# Autodesk Inventor assembly: Tube holder 1 assembly
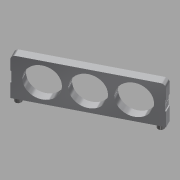
[picture p0: Inventor's stored thumbnail of the model, 180x180]
Saved by Autodesk Inventor 2017 (Build 210142000, 142)
## iProperties
Created: 2017-02-01
Part Number: Tube holder 1 assembly
Document SubType Name: Assembly
Designer: qupec
Author: qupec
## Documents named in this file (4)
- C:\Users\qupec\Desktop\UMD Near Space\RockSat\Renderings and PDFs\Tube holder 1 assembly.iam
- C:\Users\qupec\Documents\Inventor\Content Center Files\R2017\en-US\U UNC 2603(1)\Unbrako - 4 x 1 - 48 - 1 - Unbrako.ipt
- C:\Users\qupec\Desktop\UMD Near Space\RockSat\Tube Holder Halve 2.ipt
- C:\Users\qupec\Desktop\UMD Near Space\RockSat\Tube Holder Halve.ipt
## Components (4 placed, 3 different names)
1. Unbrako UNC Hex Socket Cap - Inch 4 x 1 - Unbrako:1 — Mate:1, Mate:4, Mate:6
2. Unbrako UNC Hex Socket Cap - Inch 4 x 1 - Unbrako:2 — Mate:2, Mate:3, Mate:7
3. Tube Holder Halve 2:1 — Mate:3, Mate:4, Mate:5
4. Tube Holder Halve:1 — Mate:1, Mate:2, Mate:5, Mate:6, Mate:7
## Relationships (7: Mate 7)
- Mate:1: Unbrako UNC Hex Socket Cap - Inch 4 x 1 - Unbrako:1 ↔ Tube Holder Halve:1
- Mate:2: Unbrako UNC Hex Socket Cap - Inch 4 x 1 - Unbrako:2 ↔ Tube Holder Halve:1
- Mate:3: Unbrako UNC Hex Socket Cap - Inch 4 x 1 - Unbrako:2 ↔ Tube Holder Halve 2:1
- Mate:4: Unbrako UNC Hex Socket Cap - Inch 4 x 1 - Unbrako:1 ↔ Tube Holder Halve 2:1
- Mate:5: Tube Holder Halve 2:1 ↔ Tube Holder Halve:1
- Mate:6: Unbrako UNC Hex Socket Cap - Inch 4 x 1 - Unbrako:1 ↔ Tube Holder Halve:1
- Mate:7: Unbrako UNC Hex Socket Cap - Inch 4 x 1 - Unbrako:2 ↔ Tube Holder Halve:1
